# Autodesk Inventor assembly: enc-BackPanel Unten - Assembly
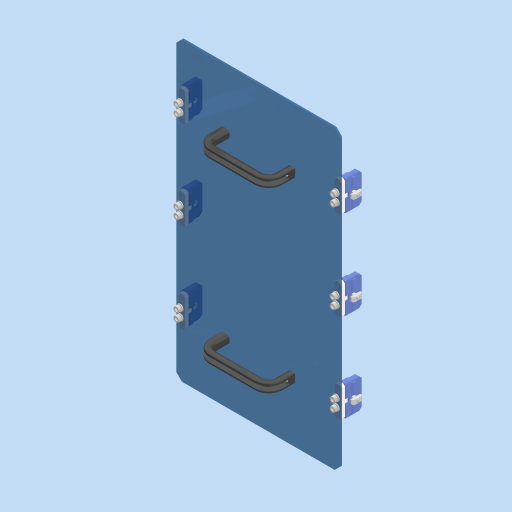
[picture p0: Inventor's stored thumbnail of the model, 512x512]
Saved by Autodesk Inventor 2023.2 (Build 272271000, 271)
## iProperties
Created: 2023-12-04
Part Number: enc-BackPanel Unten - Assembly
Document SubType Name: Assembly
Designer: Nils Bade
Author: Nils Bade
## Documents named in this file (4)
- C:\Users\nilsb\Documents\Inventor\Projektarbeit-Bade\Enclosure\enc-BackPanel Unten - Assembly.iam
- C:\Users\nilsb\Documents\Inventor\Projektarbeit-Bade\Enclosure\enc-BackPanel Unten.ipt
- C:\Users\nilsb\Documents\Inventor\Projektarbeit-Bade\Enclosure\Magnet PanelFrame 90deg connected.iam
- C:\Users\nilsb\Documents\Inventor\Projektarbeit-Bade\Enclosure\item_Handgriff_PA120_Assembly.iam
## Components (9 placed, 3 different names)
1. Magnet PanelFrame 90deg connected:1 [sub-assembly] — Passend:32, Passend:33, Passend:34
2. Magnet PanelFrame 90deg connected:2 [sub-assembly] — Passend:35, Passend:36, Passend:37
3. Magnet PanelFrame 90deg connected:3 [sub-assembly] — Passend:38, Passend:39, Passend:40
4. Magnet PanelFrame 90deg connected:4 [sub-assembly] — Passend:23, Passend:24, Passend:25
5. Magnet PanelFrame 90deg connected:5 [sub-assembly] — Passend:26, Passend:27, Passend:28
6. Magnet PanelFrame 90deg connected:6 [sub-assembly] — Passend:29, Passend:30, Passend:31
7. item_Handgriff_120er:2 [sub-assembly] — Passend:41, Passend:43, Passend:46
8. item_Handgriff_120er:1 [sub-assembly] — Passend:42, Passend:44, Passend:45
9. enc-BackPanel Unten:1 — Passend:23, Passend:24, Passend:25, Passend:26, Passend:27, Passend:28, Passend:29, Passend:30, Passend:31, Passend:32, Passend:33, Passend:34, Passend:35, Passend:36, Passend:37, Passend:38, Passend:39, Passend:40, Passend:41, Passend:42, Passend:43, Passend:44, Passend:45, Passend:46
## Relationships (24: Mate 24)
- Passend:23 [Mate]: Magnet PanelFrame 90deg connected:4 ↔ enc-BackPanel Unten:1
- Passend:24 [Mate]: Magnet PanelFrame 90deg connected:4 ↔ enc-BackPanel Unten:1
- Passend:25 [Mate]: Magnet PanelFrame 90deg connected:4 ↔ enc-BackPanel Unten:1
- Passend:26 [Mate]: Magnet PanelFrame 90deg connected:5 ↔ enc-BackPanel Unten:1
- Passend:27 [Mate]: Magnet PanelFrame 90deg connected:5 ↔ enc-BackPanel Unten:1
- Passend:28 [Mate]: Magnet PanelFrame 90deg connected:5 ↔ enc-BackPanel Unten:1
- Passend:29 [Mate]: Magnet PanelFrame 90deg connected:6 ↔ enc-BackPanel Unten:1
- Passend:30 [Mate]: Magnet PanelFrame 90deg connected:6 ↔ enc-BackPanel Unten:1
- Passend:31 [Mate]: Magnet PanelFrame 90deg connected:6 ↔ enc-BackPanel Unten:1
- Passend:32 [Mate]: Magnet PanelFrame 90deg connected:1 ↔ enc-BackPanel Unten:1
- Passend:33 [Mate]: Magnet PanelFrame 90deg connected:1 ↔ enc-BackPanel Unten:1
- Passend:34 [Mate]: Magnet PanelFrame 90deg connected:1 ↔ enc-BackPanel Unten:1
- Passend:35 [Mate]: Magnet PanelFrame 90deg connected:2 ↔ enc-BackPanel Unten:1
- Passend:36 [Mate]: Magnet PanelFrame 90deg connected:2 ↔ enc-BackPanel Unten:1
- Passend:37 [Mate]: Magnet PanelFrame 90deg connected:2 ↔ enc-BackPanel Unten:1
- Passend:38 [Mate]: Magnet PanelFrame 90deg connected:3 ↔ enc-BackPanel Unten:1
- Passend:39 [Mate]: Magnet PanelFrame 90deg connected:3 ↔ enc-BackPanel Unten:1
- Passend:40 [Mate]: Magnet PanelFrame 90deg connected:3 ↔ enc-BackPanel Unten:1
- Passend:41 [Mate]: item_Handgriff_120er:2 ↔ enc-BackPanel Unten:1
- Passend:42 [Mate]: item_Handgriff_120er:1 ↔ enc-BackPanel Unten:1
- Passend:43 [Mate]: item_Handgriff_120er:2 ↔ enc-BackPanel Unten:1
- Passend:44 [Mate]: item_Handgriff_120er:1 ↔ enc-BackPanel Unten:1
- Passend:45 [Mate]: item_Handgriff_120er:1 ↔ enc-BackPanel Unten:1
- Passend:46 [Mate]: item_Handgriff_120er:2 ↔ enc-BackPanel Unten:1
